# Autodesk Inventor assembly: AzureKinectAssembly
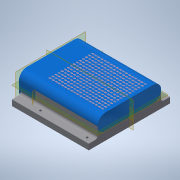
[picture p0: Inventor's stored thumbnail of the model, 180x180]
Saved by Autodesk Inventor 2020.3 (Build 243373010, 373A)
## iProperties
Created: 2020-02-21
Part Number: AzureKinectAssembly
Material: 一般
Document SubType Name: Assembly
Designer: gisen
Author: gisen
## Documents named in this file (3)
- C:\Users\gisen\GitProjects\CAD-Data\AzureKinect\AzureKinectAssembly.iam
- C:\Users\gisen\GitProjects\CAD-Data\AzureKinect\AzureKinect.ipt
- C:\Users\gisen\GitProjects\CAD-Data\AzureKinect\AzureKinectCradle.ipt
## Components (2 placed, 2 different names)
1. AzureKinect:1 — フラッシュ:1, メイト:1, メイト:2
2. AzureKinectCradle:1 — フラッシュ:1, メイト:1, メイト:2
## Relationships (3: Mate 2, Flush 1)
- フラッシュ:1 [Flush]: AzureKinect:1 ↔ AzureKinectCradle:1
- メイト:1 [Mate]: AzureKinect:1 ↔ AzureKinectCradle:1
- メイト:2 [Mate]: AzureKinect:1 ↔ AzureKinectCradle:1
